# Autodesk Inventor assembly: s-assy-pulley-j3
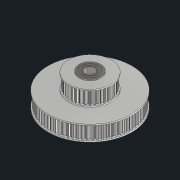
[picture p0: Inventor's stored thumbnail of the model, 180x180]
Saved by Autodesk Inventor 2021 (Build 250183000, 183)
## iProperties
Created: 2021-07-17
Part Number: s-assy-pulley-j3
Document SubType Name: Assembly
Designer: yuta0
Mass: 67.7209 g
Surface Area: 168.718 cm^2
Volume: 53.8292 cm^3
Density: 1.25807 g/cm^3
Author: yuta0
## Documents named in this file (3)
- C:\Users\yuta0\Desktop\catchrobo_robot\s-assy-pulley-j3.iam
- C:\Users\yuta0\Desktop\catchrobo_robot\base15.ipt
- C:\Users\yuta0\Desktop\catchrobo_robot\FL688ZZ.ipt
## Components (3 placed, 2 different names)
1. S3Mpully-base3:1 — メイト:1, メイト:3, メイト:4, メイト:5
2. FL688ZZ:1 — メイト:1, メイト:5
3. FL688ZZ:2 — メイト:3, メイト:4
## Relationships (4: Mate 4)
- メイト:1 [Mate]: S3Mpully-base3:1 ↔ FL688ZZ:1
- メイト:3 [Mate]: S3Mpully-base3:1 ↔ FL688ZZ:2
- メイト:4 [Mate]: S3Mpully-base3:1 ↔ FL688ZZ:2
- メイト:5 [Mate]: S3Mpully-base3:1 ↔ FL688ZZ:1
